# Autodesk Inventor assembly: car
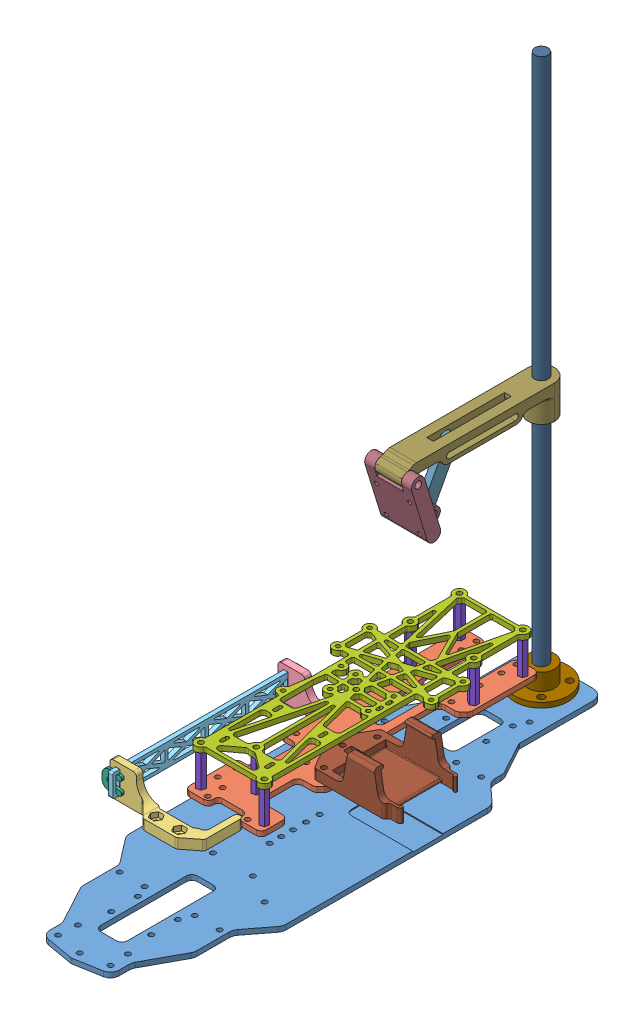
[picture p0: shaded view drawn from the shape stored in the file]
Saved by Autodesk Inventor 2021 (Build 250183000, 183)
## iProperties
Created: 2021-02-01
Part Number: car
Document SubType Name: Assembly
Designer: User
Author: User
## Documents named in this file (13)
- D:\SynologyDrive\tcodev\tco-cad\car\car.iam
- D:\SynologyDrive\tcodev\tco-cad\chassis_short\base_short.ipt
- D:\SynologyDrive\tcodev\tco-cad\chassis_short\top_short.ipt
- D:\SynologyDrive\tcodev\tco-cad\mount_battery\mount_battery.ipt
- D:\SynologyDrive\tcodev\tco-cad\mount_battery\mount_battery_mirrored.ipt
- D:\SynologyDrive\tcodev\tco-cad\mount_battery\mount_battery_fastener.ipt
- D:\SynologyDrive\tcodev\tco-cad\mount_battery\fastener_clip.ipt
- D:\SynologyDrive\tcodev\tco-cad\mount_esc\mount_esc.ipt
- D:\SynologyDrive\tcodev\tco-cad\plate_electronics\plate.ipt
- D:\SynologyDrive\tcodev\tco-cad\common\standoff_3m20mm.ipt
- D:\SynologyDrive\tcodev\tco-cad\common\flange_8mm.ipt
- D:\SynologyDrive\tcodev\tco-cad\common\rod.ipt
- D:\SynologyDrive\tcodev\tco-cad\mount_camera_manual\mount_camera_manual.iam
## Components (19 placed, 12 different names)
1. base_short:1 — Rigid:2, Rigid:3, Rigid:4, Mate:5, Mate:6, Mate:7, Angle:2
2. top_short:1 — Rigid:2, Rigid:7, Rotational:1, Rotational:2, Rotational:3, Rigid:8, Rotational:4, Rotational:5, Rotational:6, Angle:1
3. mount_battery:1 — Rigid:3, Flush:1, Mate:2
4. mount_battery_mirrored:1 — Rigid:4, Mate:1
5. mount_battery_fastener:1 — Mate:1, Flush:1, Mate:2, Rigid:5, Rigid:6
6. fastener_clip:1 — Rigid:5
7. fastener_clip:2 — Rigid:6
8. mount_esc:1 — Rigid:7
9. plate:1 — Mate:3, Mate:4, Angle:1
10. standoff_3m20mm:1 — Rotational:3
11. standoff_3m20mm:2 — Rotational:1
12. standoff_3m20mm:3 — Rigid:8
13. standoff_3m20mm:4 — Rotational:2
14. standoff_3m20mm:5 — Rotational:6
15. standoff_3m20mm:6 — Rotational:5, Mate:3, Mate:4
16. standoff_3m20mm:7 — Rotational:4
17. flange_8mm:1 — Mate:5, Mate:6, Mate:7, Mate:8, Mate:9
18. rod:1 — Mate:8, Mate:9, Mate:10
19. mount_camera_manual:1 [sub-assembly] — Mate:10, Angle:2
## Relationships (26: Mate 10, WeldJoint 7, RevoluteJoint 6, Angle 2, Flush 1)
- Rigid:2 [WeldJoint] (-28 mm): base_short:1 ↔ top_short:1
- Rigid:3 [WeldJoint]: base_short:1 ↔ mount_battery:1
- Rigid:4 [WeldJoint]: base_short:1 ↔ mount_battery_mirrored:1
- Mate:1 (0.2 mm): mount_battery_mirrored:1 ↔ mount_battery_fastener:1
- Flush:1: mount_battery:1 ↔ mount_battery_fastener:1
- Mate:2 (0.2 mm): mount_battery:1 ↔ mount_battery_fastener:1
- Rigid:5 [WeldJoint] (0.2 mm): mount_battery_fastener:1 ↔ fastener_clip:1
- Rigid:6 [WeldJoint] (0.2 mm): mount_battery_fastener:1 ↔ fastener_clip:2
- Rigid:7 [WeldJoint]: top_short:1 ↔ mount_esc:1
- Rotational:1 [RevoluteJoint]: top_short:1 ↔ standoff_3m20mm:2
- Rotational:2 [RevoluteJoint]: top_short:1 ↔ standoff_3m20mm:4
- Rotational:3 [RevoluteJoint]: top_short:1 ↔ standoff_3m20mm:1
- Rigid:8 [WeldJoint]: top_short:1 ↔ standoff_3m20mm:3
- Rotational:4 [RevoluteJoint]: top_short:1 ↔ standoff_3m20mm:7
- Rotational:5 [RevoluteJoint]: top_short:1 ↔ standoff_3m20mm:6
- Rotational:6 [RevoluteJoint]: top_short:1 ↔ standoff_3m20mm:5
- Mate:3: plate:1 ↔ standoff_3m20mm:6
- Mate:4: plate:1 ↔ standoff_3m20mm:6
- Angle:1 (0 deg): top_short:1 ↔ plate:1
- Mate:5: base_short:1 ↔ flange_8mm:1
- Mate:6: base_short:1 ↔ flange_8mm:1
- Mate:7: base_short:1 ↔ flange_8mm:1
- Mate:8: flange_8mm:1 ↔ rod:1
- Mate:9: flange_8mm:1 ↔ rod:1
- Mate:10: rod:1 ↔ mount_camera_manual:1
- Angle:2 (0 deg): base_short:1 ↔ mount_camera_manual:1
